# Autodesk Inventor assembly: ring-holder-one-sixth-2
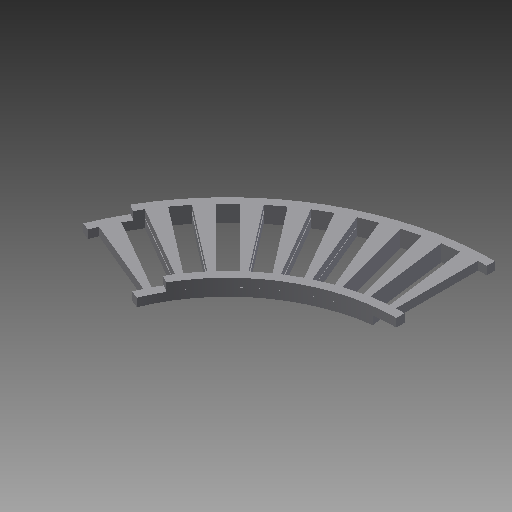
[picture p0: Inventor's stored thumbnail of the model, 512x512]
Saved by Autodesk Inventor 2018 (Build 220112000, 112)
## iProperties
Created: 2024-05-02
Part Number: ring-holder-one-sixth-2
Document SubType Name: Assembly
Designer: neo
Mass: 41.6522 g
Surface Area: 293 cm^2
Volume: 41.6522 cm^3
Density: 1 g/cm^3
Author: neo
## Documents named in this file (2)
- D:\projects\kreion\design1\3d\ring-holder-one-sixth-2.iam
- D:\projects\kreion\design1\3d\stator-60deg-holder.ipt
## Components (2 placed, 1 different names)
1. stator-60deg-holder:1 — Mate:1, Flush:1, Tangent:1
2. stator-60deg-holder:2 — Mate:1, Flush:1, Tangent:1
## Relationships (3: Mate 1, Flush 1, Tangent 1)
- Mate:1: stator-60deg-holder:1 ↔ stator-60deg-holder:2
- Flush:1: stator-60deg-holder:1 ↔ stator-60deg-holder:2
- Tangent:1: stator-60deg-holder:1 ↔ stator-60deg-holder:2
